# Autodesk Inventor assembly: wemos d1 mini V4
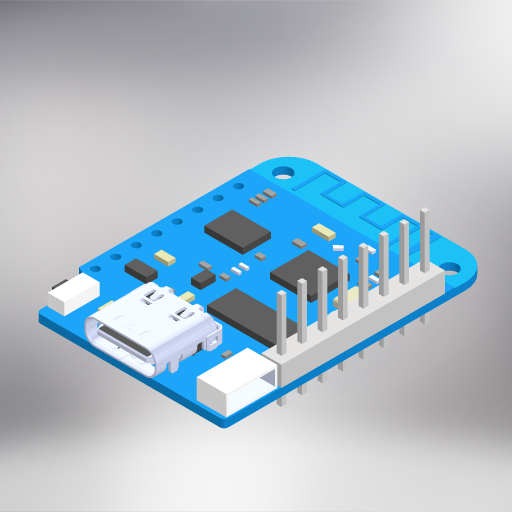
[picture p0: Inventor's stored thumbnail of the model, 512x512]
Saved by Autodesk Inventor 2024 (Build 280153000, 153)
## iProperties
Created: 2022-11-25
Part Number: wemos d1 mini V4
Description: STEP AP214
Document SubType Name: Assembly
Designer: Tejas
Sending System: SolidWorks 2020
Preprocessor: SwSTEP 2.0
Title: wemos d1 mini V4.STEP
Author: user
Revision Number: ANY
## Documents named in this file (5)
- C:\Users\Tejas\Documents\Uni 2024 T3\COMP6841\CAD\wemos d1 mini V4\wemos d1 mini V4.iam
- C:\Users\Tejas\Documents\Uni 2024 T3\COMP6841\CAD\wemos d1 mini V4\USB C + USB A 3.1.stp.ipt
- C:\Users\Tejas\Documents\Uni 2024 T3\COMP6841\CAD\wemos d1 mini V4\main board.ipt
- C:\Users\Tejas\Documents\Uni 2024 T3\COMP6841\CAD\Header D1.ipt
- USB C + USB A 3.1.stp
## Components (10 placed, 3 different names)
1. USB C + USB A 3.1.stp_1
2. main board_2 — Rigid:1, Rigid:2, Rigid:3, Rigid:4, Rigid:5, Rigid:6, Rigid:7, Rigid:8
3. Header D1:1 — Rigid:1
4. Header D1:2 — Rigid:2
5. Header D1:3 — Rigid:4
6. Header D1:4 — Rigid:3
7. Header D1:5 — Rigid:5
8. Header D1:6 — Rigid:6
9. Header D1:7 — Rigid:7
10. Header D1:8 — Rigid:8
## Relationships (8: WeldJoint 8)
- Rigid:1 [WeldJoint] (2 mm): main board_2 ↔ Header D1:1
- Rigid:2 [WeldJoint] (2 mm): main board_2 ↔ Header D1:2
- Rigid:3 [WeldJoint] (2 mm): main board_2 ↔ Header D1:4
- Rigid:4 [WeldJoint] (2 mm): main board_2 ↔ Header D1:3
- Rigid:5 [WeldJoint] (2 mm): main board_2 ↔ Header D1:5
- Rigid:6 [WeldJoint] (2 mm): main board_2 ↔ Header D1:6
- Rigid:7 [WeldJoint] (2 mm): main board_2 ↔ Header D1:7
- Rigid:8 [WeldJoint] (2 mm): main board_2 ↔ Header D1:8
